# Autodesk Inventor assembly: Buttons Mold_Remote Buttons_1_LY
Saved by Autodesk Inventor 2016 (Build 200138000, 138)
## iProperties
Created: 2015-07-01
Part Number: Buttons Mold_Remote Buttons_1_LY
Document SubType Name: Assembly
Designer: Samuel Clay
Author: Samuel Clay
## Documents named in this file (2)
- Z:\turntouch\remote\enclosure\inventor\Molds\Buttons Mold_Remote Buttons_1_LY.iam
- Z:\turntouch\remote\enclosure\inventor\Molds\Buttons Mold_Remote Buttons_1_PZ.iam
## Components (1 placed, 1 different names)
1. Buttons Mold_Remote Buttons_1_PZ:1 [sub-assembly] — Flush:1, Flush:2, Flush:3
## Relationships (3: Flush 3)
- Flush:1: Buttons Mold_Remote Buttons_1_PZ:1
- Flush:2: Buttons Mold_Remote Buttons_1_PZ:1
- Flush:3: Buttons Mold_Remote Buttons_1_PZ:1
